# Autodesk Inventor assembly: ensemble
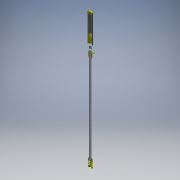
[picture p0: Inventor's stored thumbnail of the model, 180x180]
Saved by Autodesk Inventor 2019 (Build 230136000, 136)
## iProperties
Created: 2018-05-05
Part Number: ensemble
Material: Générique
Document SubType Name: Assembly
Designer: Theo
Author: Theo
## Documents named in this file (9)
- C:\dev\projects\ace\ace-git\ACE 22 A\ensemble.iam
- C:\dev\projects\ace\ace-git\ACE 22 A\support_joint.ipt
- C:\dev\projects\ace\ace-git\ACE 22 A\support_entree_air.ipt
- C:\dev\projects\ace\ace-git\ACE 22 A\douille.ipt
- C:\dev\projects\ace\ace-git\ACE 22 A\joint.ipt
- C:\dev\projects\ace\ace-git\ACE 22 A\canon_pvc.ipt
- C:\dev\projects\ace\ace-git\ACE 22 A\reservoir_pvc.ipt
- C:\dev\projects\ace\ace-git\ACE 22 A\frein_de_bouche.ipt
- C:\dev\projects\ace\ace-git\ACE 22 A\canon_support_entree.ipt
## Components (8 placed, 8 different names)
1. support_joint:1 — Placage:2, Placage:3, Placage:4, Placage:5, Placage:7, Placage:10
2. support_entree_air:1 — Placage:6, Placage:8, Placage:9
3. douille:1 — Placage:2
4. joint:1 — Placage:3
5. canon_pvc:1 — Placage:4, Placage:11, Placage:12, Placage:13, Placage:14
6. reservoir_pvc:1 — Placage:5, Placage:6, Placage:8, Placage:10
7. frein_de_bouche:1 — Placage:11, Placage:12
8. canon_support_entree:1 — Placage:13, Placage:14
## Relationships (13: Mate 13)
- Placage:2 [Mate]: support_joint:1 ↔ douille:1
- Placage:3 [Mate]: support_joint:1 ↔ joint:1
- Placage:4 [Mate]: support_joint:1 ↔ canon_pvc:1
- Placage:5 [Mate]: support_joint:1 ↔ reservoir_pvc:1
- Placage:6 [Mate]: support_entree_air:1 ↔ reservoir_pvc:1
- Placage:7 [Mate]: support_joint:1
- Placage:8 [Mate]: support_entree_air:1 ↔ reservoir_pvc:1
- Placage:9 [Mate]: support_entree_air:1
- Placage:10 [Mate]: support_joint:1 ↔ reservoir_pvc:1
- Placage:11 [Mate]: canon_pvc:1 ↔ frein_de_bouche:1
- Placage:12 [Mate]: canon_pvc:1 ↔ frein_de_bouche:1
- Placage:13 [Mate]: canon_pvc:1 ↔ canon_support_entree:1
- Placage:14 [Mate]: canon_pvc:1 ↔ canon_support_entree:1
